# Autodesk Inventor assembly: Assembly1
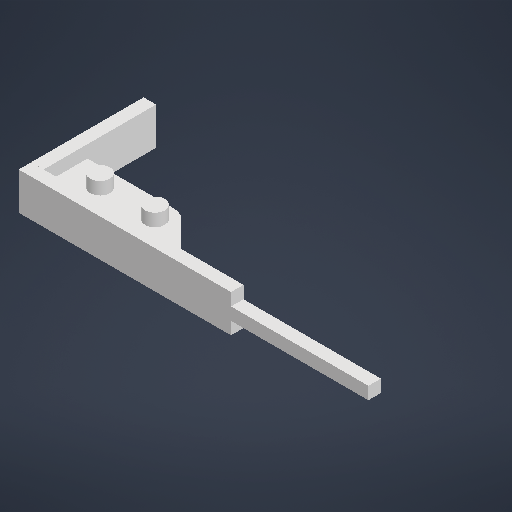
[picture p0: Inventor's stored thumbnail of the model, 512x512]
Saved by Autodesk Inventor 2026.2 (Build 302298000, 298)
## iProperties
Created: 2026-03-23
Part Number: Assembly1
Document SubType Name: Assembly
Designer: Cobble
Author: Cobble
## Documents named in this file (3)
- D:\Archive\Kreative Projekte\Obsidian\Online\Projects\Shot-Dispenser\Design V3\Part 2\Assembly1.iam
- D:\Archive\Kreative Projekte\Obsidian\Online\Projects\Shot-Dispenser\Design V3\Part 2\Basseipt.ipt
- D:\Archive\Kreative Projekte\Obsidian\Online\Projects\Shot-Dispenser\Design V3\Part 2\Basseipt_MIR.ipt
## Components (2 placed, 2 different names)
1. Basseipt:2 — Mate:1, Mate:2
2. Basseipt_MIR:1 — Mate:1, Mate:2
## Relationships (2: Mate 2)
- Mate:1: Basseipt:2 ↔ Basseipt_MIR:1
- Mate:2: Basseipt:2 ↔ Basseipt_MIR:1
